# Autodesk Inventor assembly: lower arm Assembly 800.ipt
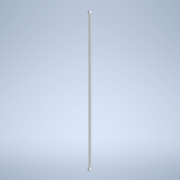
[picture p0: Inventor's stored thumbnail of the model, 180x180]
Saved by Autodesk Inventor 2021 (Build 250183000, 183)
## iProperties
Created: 2022-09-08
Part Number: lower arm Assembly 800.ipt
Document SubType Name: Assembly
Designer: szucs
Author: szucs
## Documents named in this file (3)
- C:\Users\szucs\Desktop\GTPR\ver2\lower arm Assembly 800.ipt.iam
- C:\Users\szucs\Desktop\GTPR\ver2\Rod End 8mm.iam
- C:\Users\szucs\Desktop\GTPR\ver2\lower arm 800.ipt
## Components (3 placed, 2 different names)
1. Rod End 8mm:1 [sub-assembly] — Mate:1, Mate:2, Flush:1
2. lower arm 800:1 — Mate:1, Mate:2, Mate:3, Mate:4
3. Rod End 8mm:2 [sub-assembly] — Mate:3, Mate:4, Flush:1, Angle:1
## Relationships (6: Mate 4, Flush 1, Angle 1)
- Mate:1: Rod End 8mm:1 ↔ lower arm 800:1
- Mate:2: Rod End 8mm:1 ↔ lower arm 800:1
- Mate:3: lower arm 800:1 ↔ Rod End 8mm:2
- Mate:4: lower arm 800:1 ↔ Rod End 8mm:2
- Flush:1: Rod End 8mm:1 ↔ Rod End 8mm:2
- Angle:1 (0 deg): Rod End 8mm:2
